# Autodesk Inventor assembly: FrameBoxLow
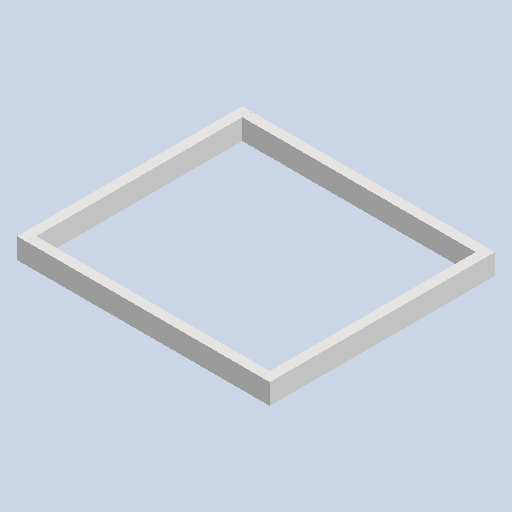
[picture p0: Inventor's stored thumbnail of the model, 512x512]
Saved by Autodesk Inventor 2023 (Build 270158000, 158)
## iProperties
Created: 2022-07-13
Part Number: FrameBoxLow
Document SubType Name: Assembly
Designer: plebbb
Author: plebbb
## Documents named in this file (3)
- D:\Users\plebbb\Desktop\CNC_Project\FrameBoxLow.iam
- D:\Users\plebbb\Desktop\CNC_Project\WOOD\2x4x41.ipt
- D:\Users\plebbb\Desktop\CNC_Project\WOOD\2x4x42.5.ipt
## Components (4 placed, 2 different names)
1. 2x4x41:1
2. 2x4x41:2
3. 2x4x42.5:1
4. 2x4x42.5:2
## Relationships (5: Flush 3, Mate 2)
- [Flush]: 2x4x41:1 ↔ 2x4x41:2
- [Mate]: 2x4x41:2 ↔ 2x4x42.5:1
- [Flush]: 2x4x41:2 ↔ 2x4x42.5:1
- [Mate]: 2x4x41:2 ↔ 2x4x42.5:2
- [Flush]: 2x4x41:1 ↔ 2x4x42.5:2
